# Autodesk Inventor assembly: электроника
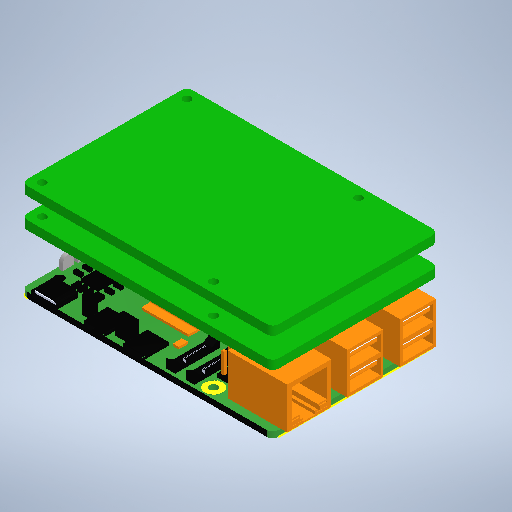
[picture p0: Inventor's stored thumbnail of the model, 512x512]
Saved by Autodesk Inventor 2025 (Build 290162000, 162)
## iProperties
Created: 2025-02-25
Part Number: электроника
Document SubType Name: Assembly
Designer: volko
Author: volko
## Documents named in this file (4)
- C:\Users\volko\Desktop\диплом\Модели\детали\электроника.iam
- C:\Users\volko\Desktop\диплом\Модели\детали\Raspberry Pi 5.ipt
- C:\Users\volko\Desktop\диплом\Модели\детали\плата двигателей.ipt
- C:\Users\volko\Desktop\диплом\Модели\детали\стандартные изделия\ru-RU\AS 1427(05)\AS 1427 - M2,5 x 25(5) II.ipt
## Components (4 placed, 3 different names)
1. Raspberry Pi 5:1 — Заподлицо:1, Заподлицо:2, Заподлицо:3
2. плата двигателей:1 — Заподлицо:4, Заподлицо:5, Заподлицо:8
3. плата двигателей:2 — Заподлицо:6, Заподлицо:7, Заподлицо:9
4. AS 1427 H - метрическая M2,5 x 25:1
## Relationships (9: Flush 9)
- Заподлицо:1 [Flush]: Raspberry Pi 5:1
- Заподлицо:2 [Flush]: Raspberry Pi 5:1
- Заподлицо:3 [Flush]: Raspberry Pi 5:1
- Заподлицо:4 [Flush]: плата двигателей:1
- Заподлицо:5 [Flush]: плата двигателей:1
- Заподлицо:6 [Flush]: плата двигателей:2
- Заподлицо:7 [Flush]: плата двигателей:2
- Заподлицо:8 [Flush] (20 mm): плата двигателей:1
- Заподлицо:9 [Flush] (30 mm): плата двигателей:2
